# Autodesk Inventor assembly: assembly
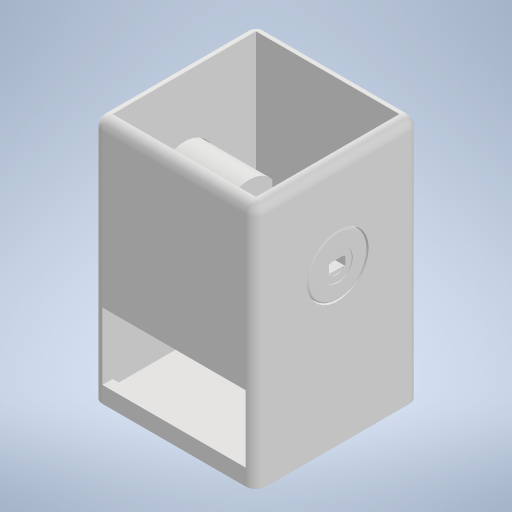
[picture p0: Inventor's stored thumbnail of the model, 512x512]
Saved by Autodesk Inventor 2024.2 (Build 282272000, 272)
## iProperties
Created: 2024-02-24
Part Number: assembly
Document SubType Name: Assembly
Designer: Luke
Author: Luke
## Documents named in this file (3)
- C:\Users\Luke\Documents\assembly.iam
- C:\Users\Luke\Documents\Dispenser.ipt
- C:\Users\Luke\Documents\spinny.ipt
## Components (2 placed, 2 different names)
1. Dispenser:1 — Mate:1, Rotational:1
2. spinny:2 — Mate:1, Rotational:1
## Relationships (2: Mate 1, RevoluteJoint 1)
- Mate:1: Dispenser:1 ↔ spinny:2
- Rotational:1 [RevoluteJoint]: Dispenser:1 ↔ spinny:2
